# Autodesk Inventor assembly: IR linear array assembly
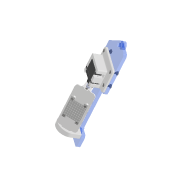
[picture p0: Inventor's stored thumbnail of the model, 180x180]
Saved by Autodesk Inventor 2020 (Build 240168000, 168)
## iProperties
Created: 2020-09-01
Part Number: IR linear array assembly
Document SubType Name: Assembly
Designer: ferrerx
Author: ferrerx
## Documents named in this file (15)
- C:\Users\ferrerx\Desktop\Prieto-Godino Lab\Drosophila Larvae Behavioural Device\Device design V3\Inventor Assembly\RGB matrices assembly.iam
- C:\Users\ferrerx\Desktop\Prieto-Godino Lab\Drosophila Larvae Behavioural Device\Device design V3\Inventor Assembly\Acrylic base light source.ipt
- C:\Users\ferrerx\Desktop\Prieto-Godino Lab\Drosophila Larvae Behavioural Device\Device design V3\Inventor Assembly\Micro servo holder.ipt
- C:\Users\ferrerx\Desktop\Prieto-Godino Lab\Drosophila Larvae Behavioural Device\Device design V3\Inventor Assembly\MG90s_servo.ipt
- C:\Users\ferrerx\Desktop\Prieto-Godino Lab\Drosophila Larvae Behavioural Device\Device design V3\Inventor Assembly\Shaft atachment.ipt
- C:\Users\ferrerx\Desktop\Prieto-Godino Lab\Drosophila Larvae Behavioural Device\Device design V3\Inventor Assembly\LED Matrix 8X8 - attachment.ipt
- C:\Users\ferrerx\Desktop\Prieto-Godino Lab\Drosophila Larvae Behavioural Device\Device design V3\Inventor Assembly\M6 spacer.ipt
- C:\Users\ferrerx\Desktop\Prieto-Godino Lab\Drosophila Larvae Behavioural Device\Device design V3\Inventor Assembly\Bearing.ipt
- C:\Users\ferrerx\Desktop\Prieto-Godino Lab\Drosophila Larvae Behavioural Device\Device design V3\Inventor Assembly\Servo lever.ipt
- C:\Users\ferrerx\Desktop\Prieto-Godino Lab\Drosophila Larvae Behavioural Device\Device design V3\Inventor Assembly\LED Matrix Dotstar.ipt
- C:\Users\ferrerx\Documents\Inventor\Content Center Files\R2020\en-US\AS 1427(04)\AS 1427 - M3 x 12(5) I.ipt
- C:\Users\ferrerx\Documents\Inventor\Content Center Files\R2020\en-US\AS 1427(04)\AS 1427 - M2 x 10(5) I.ipt
- C:\Users\ferrerx\Documents\Inventor\Content Center Files\R2020\en-US\AS 1427(04)\AS 1427 - M2 x 8(5) I.ipt
- C:\Users\ferrerx\Documents\Inventor\Content Center Files\R2020\en-US\BS 4183(1)\BS 4183 - M3(1).ipt
- C:\Users\ferrerx\Documents\Inventor\Content Center Files\R2020\en-US\BS 4183(1)\BS 4183 - M2(1).ipt
## Components (36 placed, 14 different names)
1. Acrylic base light source:1 — Mate:1, Mate:2, Mate:3, Mate:4, Mate:5, Mate:6, Mate:12, Mate:13, Mate:14, Mate:15, Mate:31
2. Micro servo holder:1 — Mate:1, Mate:2, Mate:3, Mate:8, Angle:1, Mate:9, Mate:22, Mate:23, Mate:28, Mate:29, Mate:30, Flush:4, Flush:5, Flush:6
3. MG90s_servo:1 — Mate:8, Angle:1, Mate:9, Mate:18
4. Shaft atachment:1 — Mate:4, Mate:5, Mate:6, Mate:10, Mate:11, Mate:16, Mate:17, Mate:32, Mate:33, Mate:34, Flush:1, Flush:2, Flush:3
5. LED Matrix 8X8 - attachment:1 — Mate:10, Mate:11, Mate:19, Angle:2, Mate:20, Mate:21, Angle:3, Mate:36
6. M6 spacer:1 — Mate:12, Mate:14
7. M6 spacer:2 — Mate:13, Mate:15
8. Bearing:1 — Mate:16, Mate:17
9. Servo lever:1 — Mate:18, Mate:19, Angle:2, Mate:35
10. LED Matrix Dotstar:1 — Mate:20, Mate:21, Angle:3, Mate:24, Mate:25, Mate:26, Mate:27
11. AS 1427 H - Metric M3 x 12:1 — Mate:34, Flush:1, Mate:37
12. AS 1427 H - Metric M3 x 12:2 — Mate:33, Flush:3, Mate:38
13. AS 1427 H - Metric M3 x 12:3 — Mate:32, Flush:2, Mate:39
14. AS 1427 H - Metric M3 x 12:4 — Mate:31, Mate:41
15. AS 1427 H - Metric M3 x 12:5 — Mate:30, Flush:6, Mate:42
16. AS 1427 H - Metric M3 x 12:6 — Mate:29, Flush:4, Mate:40
17. AS 1427 H - Metric M3 x 12:7 — Mate:28, Flush:5, Mate:43
18. AS 1427 H - Metric M2 x 10:1 — Mate:26, Mate:44
19. AS 1427 H - Metric M2 x 10:2 — Mate:25, Mate:45
20. AS 1427 H - Metric M2 x 10:3 — Mate:27, Mate:47
21. AS 1427 H - Metric M2 x 10:4 — Mate:24, Mate:46
22. AS 1427 H - Metric M2 x 10:5 — Mate:23
23. AS 1427 H - Metric M2 x 10:6 — Mate:22
24. AS 1427 H - Metric M2 x 8:1 — Mate:35
25. AS 1427 H - Metric M2 x 8:2 — Mate:36
26. BS 4183 - Metric M3:1 — Mate:39
27. BS 4183 - Metric M3:2 — Mate:38
28. BS 4183 - Metric M3:3 — Mate:37
29. BS 4183 - Metric M3:4 — Mate:42
30. BS 4183 - Metric M3:5 — Mate:40
31. BS 4183 - Metric M3:6 — Mate:41
32. BS 4183 - Metric M3:7 — Mate:43
33. BS 4183 - Metric M2:1 — Mate:45
34. BS 4183 - Metric M2:2 — Mate:47
35. BS 4183 - Metric M2:3 — Mate:44
36. BS 4183 - Metric M2:4 — Mate:46
## Relationships (55: Mate 46, Flush 6, Angle 3)
- Mate:1: Acrylic base light source:1 ↔ Micro servo holder:1
- Mate:2: Acrylic base light source:1 ↔ Micro servo holder:1
- Mate:3: Acrylic base light source:1 ↔ Micro servo holder:1
- Mate:4: Acrylic base light source:1 ↔ Shaft atachment:1
- Mate:5: Acrylic base light source:1 ↔ Shaft atachment:1
- Mate:6: Acrylic base light source:1 ↔ Shaft atachment:1
- Mate:8: Micro servo holder:1 ↔ MG90s_servo:1
- Angle:1 (0 deg): Micro servo holder:1 ↔ MG90s_servo:1
- Mate:9: Micro servo holder:1 ↔ MG90s_servo:1
- Mate:10: Shaft atachment:1 ↔ LED Matrix 8X8 - attachment:1
- Mate:11 (1 mm): Shaft atachment:1 ↔ LED Matrix 8X8 - attachment:1
- Mate:12: Acrylic base light source:1 ↔ M6 spacer:1
- Mate:13: Acrylic base light source:1 ↔ M6 spacer:2
- Mate:14: Acrylic base light source:1 ↔ M6 spacer:1
- Mate:15: Acrylic base light source:1 ↔ M6 spacer:2
- Mate:16: Shaft atachment:1 ↔ Bearing:1
- Mate:17: Shaft atachment:1 ↔ Bearing:1
- Mate:18: MG90s_servo:1 ↔ Servo lever:1
- Mate:19: LED Matrix 8X8 - attachment:1 ↔ Servo lever:1
- Angle:2 (0 deg): LED Matrix 8X8 - attachment:1 ↔ Servo lever:1
- Mate:20: LED Matrix 8X8 - attachment:1 ↔ LED Matrix Dotstar:1
- Mate:21: LED Matrix 8X8 - attachment:1 ↔ LED Matrix Dotstar:1
- Angle:3 (0 deg): LED Matrix 8X8 - attachment:1 ↔ LED Matrix Dotstar:1
- Mate:22: Micro servo holder:1 ↔ AS 1427 H - Metric M2 x 10:6
- Mate:23: Micro servo holder:1 ↔ AS 1427 H - Metric M2 x 10:5
- Mate:24: LED Matrix Dotstar:1 ↔ AS 1427 H - Metric M2 x 10:4
- Mate:25: LED Matrix Dotstar:1 ↔ AS 1427 H - Metric M2 x 10:2
- Mate:26: LED Matrix Dotstar:1 ↔ AS 1427 H - Metric M2 x 10:1
- Mate:27: LED Matrix Dotstar:1 ↔ AS 1427 H - Metric M2 x 10:3
- Mate:28: Micro servo holder:1 ↔ AS 1427 H - Metric M3 x 12:7
- Mate:29: Micro servo holder:1 ↔ AS 1427 H - Metric M3 x 12:6
- Mate:30: Micro servo holder:1 ↔ AS 1427 H - Metric M3 x 12:5
- Mate:31: Acrylic base light source:1 ↔ AS 1427 H - Metric M3 x 12:4
- Mate:32: Shaft atachment:1 ↔ AS 1427 H - Metric M3 x 12:3
- Mate:33: Shaft atachment:1 ↔ AS 1427 H - Metric M3 x 12:2
- Mate:34: Shaft atachment:1 ↔ AS 1427 H - Metric M3 x 12:1
- Flush:1: Shaft atachment:1 ↔ AS 1427 H - Metric M3 x 12:1
- Flush:2: Shaft atachment:1 ↔ AS 1427 H - Metric M3 x 12:3
- Flush:3: Shaft atachment:1 ↔ AS 1427 H - Metric M3 x 12:2
- Flush:4: Micro servo holder:1 ↔ AS 1427 H - Metric M3 x 12:6
- Flush:5: Micro servo holder:1 ↔ AS 1427 H - Metric M3 x 12:7
- Flush:6: Micro servo holder:1 ↔ AS 1427 H - Metric M3 x 12:5
- Mate:35: Servo lever:1 ↔ AS 1427 H - Metric M2 x 8:1
- Mate:36: LED Matrix 8X8 - attachment:1 ↔ AS 1427 H - Metric M2 x 8:2
- Mate:37: AS 1427 H - Metric M3 x 12:1 ↔ BS 4183 - Metric M3:3
- Mate:38: AS 1427 H - Metric M3 x 12:2 ↔ BS 4183 - Metric M3:2
- Mate:39: AS 1427 H - Metric M3 x 12:3 ↔ BS 4183 - Metric M3:1
- Mate:40: AS 1427 H - Metric M3 x 12:6 ↔ BS 4183 - Metric M3:5
- Mate:41: AS 1427 H - Metric M3 x 12:4 ↔ BS 4183 - Metric M3:6
- Mate:42: AS 1427 H - Metric M3 x 12:5 ↔ BS 4183 - Metric M3:4
- Mate:43: AS 1427 H - Metric M3 x 12:7 ↔ BS 4183 - Metric M3:7
- Mate:44: AS 1427 H - Metric M2 x 10:1 ↔ BS 4183 - Metric M2:3
- Mate:45: AS 1427 H - Metric M2 x 10:2 ↔ BS 4183 - Metric M2:1
- Mate:46: AS 1427 H - Metric M2 x 10:4 ↔ BS 4183 - Metric M2:4
- Mate:47: AS 1427 H - Metric M2 x 10:3 ↔ BS 4183 - Metric M2:2
